# Autodesk Inventor assembly: new collector mount
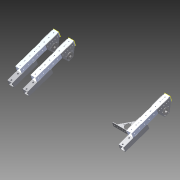
[picture p0: Inventor's stored thumbnail of the model, 180x180]
Saved by Autodesk Inventor 2014 (Build 180170000, 170)
## iProperties
Created: 2014-01-17
Part Number: new collector mount
Document SubType Name: Assembly
Designer: Arpan
Author: Arpan
## Documents named in this file (7)
- C:\Users\Michael\Documents\GitHub\2014buildCAD\new collector mount\new collector mount.iam
- C:\Users\Michael\Documents\GitHub\2014buildCAD\new collector mount\Vex Pro 1x1 rectangular tubing 9 in length.ipt
- C:\Users\Michael\Documents\GitHub\2014buildCAD\new collector mount\Vex Pro Side Bearing Gusset.ipt
- C:\Users\Michael\Documents\GitHub\2014buildCAD\new collector mount\Vex Pro Corner Gusset.ipt
- C:\Users\Michael\Documents\GitHub\2014buildCAD\New Collector\Hex Bearing 1-2 in (FR8ZZ-Hex, am-0279).ipt
- C:\Users\Michael\Documents\GitHub\2014buildCAD\new collector mount\Square Tube 1-16 thick Support.ipt
- C:\Users\Michael\Documents\GitHub\2014buildCAD\new collector mount\Vex Pro 1x1 rectangular tubing 8 in length (modified).ipt
## Components (19 placed, 6 different names)
1. Vex Pro 1x1 rectangular tubing 9 in length:1 — Mate:1, Flush:1, Flush:2, Mate:10, Mate:13, Mate:17, Mate:18, Mate:19, Mate:40, Mate:41, Mate:42, Mate:43, Mate:48, Mate:65, Mate:66
2. Vex Pro 1x1 rectangular tubing 9 in length:2 — Mate:1, Flush:1, Flush:2, Mate:4, Mate:7, Mate:36, Mate:37, Mate:38, Mate:39, Mate:45, Mate:46, Mate:47, Mate:54, Flush:7
3. Vex Pro Side Bearing Gusset:1 — Mate:4, Mate:24, Mate:25, Mate:38, Mate:39
4. Vex Pro Side Bearing Gusset:2 — Mate:7, Mate:26, Mate:27, Mate:36, Mate:37
5. Vex Pro Side Bearing Gusset:3 — Mate:10, Mate:20, Mate:21, Mate:42, Mate:43
6. Vex Pro Side Bearing Gusset:4 — Mate:13, Mate:22, Mate:23, Mate:40, Mate:41
7. Vex Pro Corner Gusset:2 — Mate:17, Mate:18, Mate:19
8. Hex Bearing 1-2 in (FR8ZZ-Hex, am-0279):1 — Mate:20, Mate:21, Flush:4, Flush:5
9. Hex Bearing 1-2 in (FR8ZZ-Hex, am-0279):2 — Mate:22, Mate:23, Flush:4
10. Hex Bearing 1-2 in (FR8ZZ-Hex, am-0279):3 — Mate:24, Mate:25, Flush:3
11. Hex Bearing 1-2 in (FR8ZZ-Hex, am-0279):4 — Mate:26, Mate:27, Flush:3, Flush:5
12. Square Tube 1-16 thick Support:1 — Mate:45, Mate:46, Mate:47, Flush:6
13. Square Tube 1-16 thick Support:2 — Mate:48, Mate:65, Mate:66
14. Square Tube 1-16 thick Support:3 — Flush:6, Mate:51, Mate:52, Mate:53
15. Vex Pro 1x1 rectangular tubing 8 in length (modified):1 — Mate:51, Mate:52, Mate:53, Mate:54, Flush:7, Mate:55, Mate:56, Mate:57, Mate:58, Mate:59, Mate:60
16. Vex Pro Side Bearing Gusset:5 — Mate:55, Mate:56, Mate:57, Mate:62, Mate:64
17. Vex Pro Side Bearing Gusset:6 — Mate:58, Mate:59, Mate:60, Mate:61, Mate:63
18. Hex Bearing 1-2 in (FR8ZZ-Hex, am-0279):5 — Mate:62, Mate:64
19. Hex Bearing 1-2 in (FR8ZZ-Hex, am-0279):6 — Mate:61, Mate:63
## Relationships (51: Mate 44, Flush 7)
- Mate:1 (533.4 mm): Vex Pro 1x1 rectangular tubing 9 in length:1 ↔ Vex Pro 1x1 rectangular tubing 9 in length:2
- Flush:1: Vex Pro 1x1 rectangular tubing 9 in length:1 ↔ Vex Pro 1x1 rectangular tubing 9 in length:2
- Flush:2: Vex Pro 1x1 rectangular tubing 9 in length:1 ↔ Vex Pro 1x1 rectangular tubing 9 in length:2
- Mate:4: Vex Pro 1x1 rectangular tubing 9 in length:2 ↔ Vex Pro Side Bearing Gusset:1
- Mate:7: Vex Pro 1x1 rectangular tubing 9 in length:2 ↔ Vex Pro Side Bearing Gusset:2
- Mate:10: Vex Pro 1x1 rectangular tubing 9 in length:1 ↔ Vex Pro Side Bearing Gusset:3
- Mate:13: Vex Pro 1x1 rectangular tubing 9 in length:1 ↔ Vex Pro Side Bearing Gusset:4
- Mate:17: Vex Pro 1x1 rectangular tubing 9 in length:1 ↔ Vex Pro Corner Gusset:2
- Mate:18: Vex Pro 1x1 rectangular tubing 9 in length:1 ↔ Vex Pro Corner Gusset:2
- Mate:19: Vex Pro 1x1 rectangular tubing 9 in length:1 ↔ Vex Pro Corner Gusset:2
- Mate:20: Vex Pro Side Bearing Gusset:3 ↔ Hex Bearing 1-2 in (FR8ZZ-Hex, am-0279):1
- Mate:21: Vex Pro Side Bearing Gusset:3 ↔ Hex Bearing 1-2 in (FR8ZZ-Hex, am-0279):1
- Mate:22: Vex Pro Side Bearing Gusset:4 ↔ Hex Bearing 1-2 in (FR8ZZ-Hex, am-0279):2
- Mate:23: Vex Pro Side Bearing Gusset:4 ↔ Hex Bearing 1-2 in (FR8ZZ-Hex, am-0279):2
- Mate:24: Vex Pro Side Bearing Gusset:1 ↔ Hex Bearing 1-2 in (FR8ZZ-Hex, am-0279):3
- Mate:25: Vex Pro Side Bearing Gusset:1 ↔ Hex Bearing 1-2 in (FR8ZZ-Hex, am-0279):3
- Mate:26: Vex Pro Side Bearing Gusset:2 ↔ Hex Bearing 1-2 in (FR8ZZ-Hex, am-0279):4
- Mate:27: Vex Pro Side Bearing Gusset:2 ↔ Hex Bearing 1-2 in (FR8ZZ-Hex, am-0279):4
- Flush:3: Hex Bearing 1-2 in (FR8ZZ-Hex, am-0279):3 ↔ Hex Bearing 1-2 in (FR8ZZ-Hex, am-0279):4
- Flush:4: Hex Bearing 1-2 in (FR8ZZ-Hex, am-0279):1 ↔ Hex Bearing 1-2 in (FR8ZZ-Hex, am-0279):2
- Flush:5: Hex Bearing 1-2 in (FR8ZZ-Hex, am-0279):1 ↔ Hex Bearing 1-2 in (FR8ZZ-Hex, am-0279):4
- Mate:36: Vex Pro 1x1 rectangular tubing 9 in length:2 ↔ Vex Pro Side Bearing Gusset:2
- Mate:37: Vex Pro 1x1 rectangular tubing 9 in length:2 ↔ Vex Pro Side Bearing Gusset:2
- Mate:38: Vex Pro 1x1 rectangular tubing 9 in length:2 ↔ Vex Pro Side Bearing Gusset:1
- Mate:39: Vex Pro 1x1 rectangular tubing 9 in length:2 ↔ Vex Pro Side Bearing Gusset:1
- Mate:40: Vex Pro 1x1 rectangular tubing 9 in length:1 ↔ Vex Pro Side Bearing Gusset:4
- Mate:41: Vex Pro 1x1 rectangular tubing 9 in length:1 ↔ Vex Pro Side Bearing Gusset:4
- Mate:42: Vex Pro 1x1 rectangular tubing 9 in length:1 ↔ Vex Pro Side Bearing Gusset:3
- Mate:43: Vex Pro 1x1 rectangular tubing 9 in length:1 ↔ Vex Pro Side Bearing Gusset:3
- Mate:45: Vex Pro 1x1 rectangular tubing 9 in length:2 ↔ Square Tube 1-16 thick Support:1
- Mate:46: Vex Pro 1x1 rectangular tubing 9 in length:2 ↔ Square Tube 1-16 thick Support:1
- Mate:47: Vex Pro 1x1 rectangular tubing 9 in length:2 ↔ Square Tube 1-16 thick Support:1
- Mate:48: Vex Pro 1x1 rectangular tubing 9 in length:1 ↔ Square Tube 1-16 thick Support:2
- Flush:6: Square Tube 1-16 thick Support:1 ↔ Square Tube 1-16 thick Support:3
- Mate:51: Square Tube 1-16 thick Support:3 ↔ Vex Pro 1x1 rectangular tubing 8 in length (modified):1
- Mate:52: Square Tube 1-16 thick Support:3 ↔ Vex Pro 1x1 rectangular tubing 8 in length (modified):1
- Mate:53: Square Tube 1-16 thick Support:3 ↔ Vex Pro 1x1 rectangular tubing 8 in length (modified):1
- Mate:54 (50.8 mm): Vex Pro 1x1 rectangular tubing 9 in length:2 ↔ Vex Pro 1x1 rectangular tubing 8 in length (modified):1
- Flush:7: Vex Pro 1x1 rectangular tubing 9 in length:2 ↔ Vex Pro 1x1 rectangular tubing 8 in length (modified):1
- Mate:55: Vex Pro 1x1 rectangular tubing 8 in length (modified):1 ↔ Vex Pro Side Bearing Gusset:5
- Mate:56: Vex Pro 1x1 rectangular tubing 8 in length (modified):1 ↔ Vex Pro Side Bearing Gusset:5
- Mate:57: Vex Pro 1x1 rectangular tubing 8 in length (modified):1 ↔ Vex Pro Side Bearing Gusset:5
- Mate:58: Vex Pro 1x1 rectangular tubing 8 in length (modified):1 ↔ Vex Pro Side Bearing Gusset:6
- Mate:59: Vex Pro 1x1 rectangular tubing 8 in length (modified):1 ↔ Vex Pro Side Bearing Gusset:6
- Mate:60: Vex Pro 1x1 rectangular tubing 8 in length (modified):1 ↔ Vex Pro Side Bearing Gusset:6
- Mate:61: Vex Pro Side Bearing Gusset:6 ↔ Hex Bearing 1-2 in (FR8ZZ-Hex, am-0279):6
- Mate:62: Vex Pro Side Bearing Gusset:5 ↔ Hex Bearing 1-2 in (FR8ZZ-Hex, am-0279):5
- Mate:63: Vex Pro Side Bearing Gusset:6 ↔ Hex Bearing 1-2 in (FR8ZZ-Hex, am-0279):6
- Mate:64: Vex Pro Side Bearing Gusset:5 ↔ Hex Bearing 1-2 in (FR8ZZ-Hex, am-0279):5
- Mate:65: Vex Pro 1x1 rectangular tubing 9 in length:1 ↔ Square Tube 1-16 thick Support:2
- Mate:66: Vex Pro 1x1 rectangular tubing 9 in length:1 ↔ Square Tube 1-16 thick Support:2
